# Autodesk Inventor assembly: 部件1
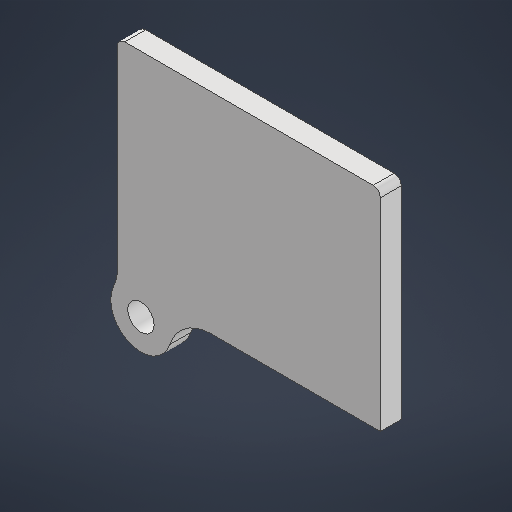
[picture p0: Inventor's stored thumbnail of the model, 512x512]
Saved by Autodesk Inventor 2025 (Build 290162000, 162)
## iProperties
Created: 2025-11-30
Part Number: 部件1
Document SubType Name: Assembly
Designer: XH
Author: XH
## Documents named in this file (3)
- C:\1A_Engineering_files\Samsung_zflip5\部件1.iam
- C:\1A_Engineering_files\Samsung_zflip5\电子\键盘.ipt
- C:\1A_Engineering_files\Samsung_zflip5\真键盘外壳.ipt
## Components (2 placed, 2 different names)
1. 键盘:1 — 配合:1
2. 真键盘外壳:1 — 配合:1
## Relationships (1: Mate 1)
- 配合:1 [Mate]: 键盘:1 ↔ 真键盘外壳:1
